# Autodesk Inventor assembly: 30-0011
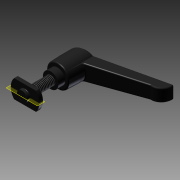
[picture p0: Inventor's stored thumbnail of the model, 180x180]
Saved by Autodesk Inventor 2011 SP2 (Build 150309200, 309)
## iProperties
Created: 2007-02-28
Part Number: 30-0011
Document SubType Name: Assembly
Designer: Raub
Manufacturer: Standard
Standards Organization: Custom
Mass: 24.6091 g
Surface Area: 68.895 cm^2
Volume: 16.6681 cm^3
Density: 1.47642 g/cm^3
Author: Raub
## Documents named in this file (3)
- R:\PSD 3 Library Update\IPS Part Files\08-Linear Application\04-Slide Block Accessories\01-Clamp Accessories\30-0011.iam
- R:\PSD 3 Library Update\IPS Part Files\08-Linear Application\04-Slide Block Accessories\01-Clamp Accessories\23-325.ipt
- R:\PSD 3 Library Update\IPS Part Files\08-Linear Application\04-Slide Block Accessories\01-Clamp Accessories\20-081.ipt
## Components (2 placed, 2 different names)
1. 23-325:1 — Insert:2
2. 20-081:1 — Insert:2
## Relationships (1: Insert 1)
- Insert:2: 23-325:1 ↔ 20-081:1
